# Autodesk Inventor assembly: Anglerfish_bonne_mamman_m12large_flipped_v0
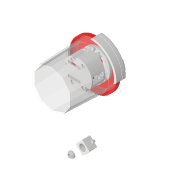
[picture p0: Inventor's stored thumbnail of the model, 180x180]
Saved by Autodesk Inventor 2022 (Build 260153000, 153)
## iProperties
Created: 2022-04-02
Part Number: Anglerfish_bonne_mamman_m12large_flipped_v0
Document SubType Name: Assembly
Designer: Prakash Lab
Author: Prakash Lab
## Documents named in this file (14)
- C:\Users\UC2\Documents\GitHub\Matchboxscope\INVENTOR\ANGLERFISH\Anglerfish_bonne_mamman_m12large_flipped_v0.iam
- C:\Users\UC2\Documents\GitHub\Matchboxscope\INVENTOR\ANGLERFISH\00_ESP3-CAM.iam
- C:\Users\UC2\Documents\GitHub\Matchboxscope\INVENTOR\ANGLERFISH\00_Powerbank.ipt
- C:\Users\diederichbenedict\Documents\Inventor\Content Center Files\R2022\de-DE\DIN 912\DIN 912 - M3 x 0.5 x 25 x 18.ipt
- C:\Users\UC2\Documents\GitHub\Matchboxscope\INVENTOR\ANGLERFISH\00_bonne_maman_jar.ipt
- C:\Users\UC2\Documents\GitHub\Matchboxscope\INVENTOR\ANGLERFISH\Matchboxscope_M12_Lensadapter_v0.ipt
- C:\Users\UC2\Documents\GitHub\Matchboxscope\INVENTOR\ANGLERFISH\00_toslink_launcher_v3.ipt
- C:\Users\UC2\Documents\GitHub\Matchboxscope\INVENTOR\ANGLERFISH\00_CCTV_M12_VCM_large.ipt
- C:\Users\UC2\Documents\GitHub\Matchboxscope\INVENTOR\ANGLERFISH\Anglerfish_flipped_LidMoun.ipt
- C:\Users\UC2\Documents\GitHub\Matchboxscope\INVENTOR\ANGLERFISH\Anglerfish_flipped_Baselayer.ipt
- C:\Users\UC2\Documents\GitHub\Matchboxscope\INVENTOR\ANGLERFISH\Anglerfish_flipped_Electronicsmount.ipt
- C:\Users\UC2\Documents\GitHub\Matchboxscope\INVENTOR\ANGLERFISH\00_Coverglass.ipt
- C:\Users\UC2\Documents\GitHub\Matchboxscope\INVENTOR\ANGLERFISH\00_Lid_Bonne_Mamman.ipt
- C:\Users\UC2\Documents\GitHub\Matchboxscope\INVENTOR\ANGLERFISH\Anglerfish_Lightplate_Tosslink_flipped.ipt
## Components (15 placed, 13 different names)
1. DIN 912 - ersetzt durch DIN EN ISO 4762 M3 x 25:5
2. DIN 912 - ersetzt durch DIN EN ISO 4762 M3 x 25:7
3. DIN 912 - ersetzt durch DIN EN ISO 4762 M3 x 25:8
4. 00_Powerbank:1
5. 00_toslink_launcher_v3:1 — Passend:28, Passend:29, Winkel:14
6. 00_bonne_maman_jar:1 — Passend:10, Winkel:1, Fluchtend:1
7. 00_ESP3-CAM:1 [sub-assembly] — Passend:23, Passend:24, Winkel:9, Winkel:11
8. 00_CCTV_M12_VCM_large:1
9. Matchboxscope_M12_Lensadapter_v0:1
10. Anglerfish_flipped_Electronicsmount:1 — Einfügen:2, Winkel:11
11. Anglerfish_flipped_LidMoun:1 — Einfügen:3
12. Anglerfish_flipped_Baselayer:1 — Passend:23, Passend:24, Winkel:9, Einfügen:2, Winkel:10
13. 00_Coverglass:1 — Passend:25, Passend:26, Winkel:13, Fluchtend:2
14. 00_Lid_Bonne_Mamman:1 — Einfügen:3, Winkel:12, Passend:25, Passend:26, Einfügen:4, Passend:27, Passend:29
15. Anglerfish_Lightplate_Tosslink_flipped:1 — Einfügen:4, Winkel:13, Passend:27, Fluchtend:2, Passend:28, Winkel:14
## Relationships (21: Mate 8, Angle 8, Insert 3, Flush 2)
- Passend:10 [Mate]: 00_bonne_maman_jar:1
- Winkel:1 [Angle] (0 deg): 00_bonne_maman_jar:1
- Fluchtend:1 [Flush]: 00_bonne_maman_jar:1
- [Angle] (45 deg): Anglerfish_flipped_Electronicsmount:1 ↔ Anglerfish_flipped_LidMoun:1
- Passend:23 [Mate]: 00_ESP3-CAM:1 ↔ Anglerfish_flipped_Baselayer:1
- Passend:24 [Mate]: 00_ESP3-CAM:1 ↔ Anglerfish_flipped_Baselayer:1
- Winkel:9 [Angle] (180 deg): 00_ESP3-CAM:1 ↔ Anglerfish_flipped_Baselayer:1
- Einfügen:2 [Insert]: Anglerfish_flipped_Electronicsmount:1 ↔ Anglerfish_flipped_Baselayer:1
- Winkel:10 [Angle] (180 deg): Anglerfish_flipped_Baselayer:1
- Winkel:11 [Angle] (180 deg): 00_ESP3-CAM:1 ↔ Anglerfish_flipped_Electronicsmount:1
- Einfügen:3 [Insert]: Anglerfish_flipped_LidMoun:1 ↔ 00_Lid_Bonne_Mamman:1
- Winkel:12 [Angle] (0 deg): 00_Lid_Bonne_Mamman:1
- Passend:25 [Mate]: 00_Coverglass:1 ↔ 00_Lid_Bonne_Mamman:1
- Passend:26 [Mate]: 00_Coverglass:1 ↔ 00_Lid_Bonne_Mamman:1
- Einfügen:4 [Insert] (1 mm): 00_Lid_Bonne_Mamman:1 ↔ Anglerfish_Lightplate_Tosslink_flipped:1
- Winkel:13 [Angle] (180 deg): 00_Coverglass:1 ↔ Anglerfish_Lightplate_Tosslink_flipped:1
- Passend:27 [Mate]: 00_Lid_Bonne_Mamman:1 ↔ Anglerfish_Lightplate_Tosslink_flipped:1
- Fluchtend:2 [Flush]: 00_Coverglass:1 ↔ Anglerfish_Lightplate_Tosslink_flipped:1
- Passend:28 [Mate]: 00_toslink_launcher_v3:1 ↔ Anglerfish_Lightplate_Tosslink_flipped:1
- Passend:29 [Mate]: 00_toslink_launcher_v3:1 ↔ 00_Lid_Bonne_Mamman:1
- Winkel:14 [Angle] (0 deg): 00_toslink_launcher_v3:1 ↔ Anglerfish_Lightplate_Tosslink_flipped:1
